# Autodesk Inventor assembly: caster_wheel_1_short
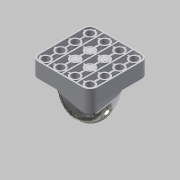
[picture p0: Inventor's stored thumbnail of the model, 180x180]
Saved by Autodesk Inventor 2019.3 (Build 233278000, 278)
## iProperties
Created: 2019-02-11
Part Number: caster_wheel_1_short
Description: STEP AP214
Document SubType Name: Assembly
Designer: Varga Daniel
Title: caster_wheel.STEP
Revision Number: ANY
Sending System: SolidWorks 2018
Preprocessor: SwSTEP 2.0
## Documents named in this file (6)
- C:\!_Dani\!_cloud\OneDrive\!_munka\Revolution\RevvyDemoKit\Structural parts\Demo parts\Caster wheel\Inventor imported\caster_wheel_1\caster_wheel_1_short.iam
- C:\!_Dani\!_cloud\OneDrive\!_munka\Revolution\RevvyDemoKit\Structural parts\Demo parts\Caster wheel\Inventor imported\caster_wheel_base.ipt
- C:\!_Dani\!_cloud\OneDrive\!_munka\Revolution\RevvyDemoKit\Structural parts\Demo parts\Caster wheel\Inventor imported\caster wheel v5.iam
- C:\!_Dani\!_cloud\OneDrive\!_munka\Revolution\RevvyDemoKit\Structural parts\Demo parts\Caster wheel\Inventor imported\Caster_wheel_inner_plug_1.ipt
- C:\!_Dani\!_cloud\OneDrive\!_munka\Revolution\RevvyDemoKit\Structural parts\Demo parts\Caster wheel\Inventor imported\caster_wheel_1.iam
- C:\!_Dani\!_cloud\OneDrive\!_munka\Revolution\RevvyDemoKit\Structural parts\Demo parts\Caster wheel\Inventor imported\Caster_wheel_inner_plug_1\Caster_wheel_inner_plug_1_01.ipt
## Components (3 placed, 3 different names)
1. caster_wheel_base_1 — Mate:2, Mate:3, Mate:5, Mate:6, Mate:7
2. caster wheel v5:1 [sub-assembly] — Mate:2, Mate:3, Angle:1, Tangent:1, Mate:4
3. Caster_wheel_inner_plug_1_01:1 — Mate:4, Mate:5, Mate:6, Mate:7
## Relationships (8: Mate 6, Angle 1, Tangent 1)
- Mate:2: caster_wheel_base_1 ↔ caster wheel v5:1
- Mate:3: caster_wheel_base_1 ↔ caster wheel v5:1
- Angle:1 (0 deg): caster wheel v5:1
- Tangent:1: caster wheel v5:1
- Mate:4: caster wheel v5:1 ↔ Caster_wheel_inner_plug_1_01:1
- Mate:5: caster_wheel_base_1 ↔ Caster_wheel_inner_plug_1_01:1
- Mate:6: caster_wheel_base_1 ↔ Caster_wheel_inner_plug_1_01:1
- Mate:7: caster_wheel_base_1 ↔ Caster_wheel_inner_plug_1_01:1
